# Autodesk Inventor assembly: ExampleServoAssembly
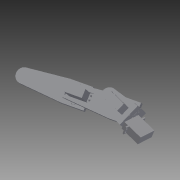
[picture p0: Inventor's stored thumbnail of the model, 180x180]
Saved by Autodesk Inventor 2014 SP1 (Build 180222100, 222)
## iProperties
Created: 2014-01-19
Part Number: ExampleServoAssembly
Document SubType Name: Assembly
Designer: david
Author: david
## Documents named in this file (6)
- C:\Users\asus\Documents\Autodesk\Projects\SheepWarrior\SheepBot.iam
- C:\Users\asus\Documents\Autodesk\Projects\RobotsWar\Docs\3D\CommonComponents\SimplifiedServo.ipt
- C:\Users\asus\Documents\Autodesk\Projects\RobotsWar\Docs\3D\CommonComponents\SimplifiedServoArm.ipt
- C:\Users\asus\Documents\Autodesk\Projects\SheepWarrior\LegParts\FrontLowerLeg.ipt
- C:\Users\asus\Documents\Autodesk\Projects\SheepWarrior\LegParts\FrontUpperLeg.ipt
- C:\Users\asus\Documents\Autodesk\Projects\SheepWarrior\LegParts\FrontUpperLegShoulder.ipt
## Components (9 placed, 5 different names)
1. SimplifiedServo:1 — Rotational:1, Insert:1, Mate:7, Mate:8, Mate:9
2. SimplifiedServoArm:1 — Rotational:1, Mate:1, Angle:1
3. FrontLowerLeg:1 — Mate:1, Insert:1, Angle:1
4. FrontUpperLeg:1 — Mate:5, Mate:6, Angle:2, Mate:7, Mate:8, Mate:9
5. SimplifiedServoArm:2 — Mate:5, Mate:6, Angle:2, Rotational:2
6. SimplifiedServo:2 — Rotational:2, Mate:10, Mate:11, Mate:12
7. FrontUpperLegShoulder:1 — Mate:10, Mate:11, Mate:12, Mate:13, Mate:14, Angle:3
8. SimplifiedServoArm:3 — Rotational:3, Mate:13, Mate:14, Angle:3
9. SimplifiedServo:3 — Rotational:3
## Relationships (18: Mate 11, RevoluteJoint 3, Angle 3, Insert 1)
- Rotational:1 [RevoluteJoint]: SimplifiedServo:1 ↔ SimplifiedServoArm:1
- Mate:1: SimplifiedServoArm:1 ↔ FrontLowerLeg:1
- Insert:1: SimplifiedServo:1 ↔ FrontLowerLeg:1
- Angle:1 (0 deg): SimplifiedServoArm:1 ↔ FrontLowerLeg:1
- Mate:5: FrontUpperLeg:1 ↔ SimplifiedServoArm:2
- Mate:6: FrontUpperLeg:1 ↔ SimplifiedServoArm:2
- Angle:2 (0 deg): FrontUpperLeg:1 ↔ SimplifiedServoArm:2
- Rotational:2 [RevoluteJoint]: SimplifiedServoArm:2 ↔ SimplifiedServo:2
- Mate:7: SimplifiedServo:1 ↔ FrontUpperLeg:1
- Mate:8: SimplifiedServo:1 ↔ FrontUpperLeg:1
- Mate:9: SimplifiedServo:1 ↔ FrontUpperLeg:1
- Mate:10: SimplifiedServo:2 ↔ FrontUpperLegShoulder:1
- Mate:11: SimplifiedServo:2 ↔ FrontUpperLegShoulder:1
- Mate:12: SimplifiedServo:2 ↔ FrontUpperLegShoulder:1
- Rotational:3 [RevoluteJoint]: SimplifiedServoArm:3 ↔ SimplifiedServo:3
- Mate:13: FrontUpperLegShoulder:1 ↔ SimplifiedServoArm:3
- Mate:14: FrontUpperLegShoulder:1 ↔ SimplifiedServoArm:3
- Angle:3 (0 deg): FrontUpperLegShoulder:1 ↔ SimplifiedServoArm:3
